# Autodesk Inventor assembly: BaseBotNoMod
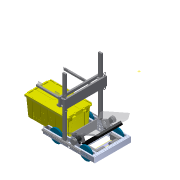
[picture p0: Inventor's stored thumbnail of the model, 180x180]
Saved by Autodesk Inventor 2015 (Build 190159000, 159)
## iProperties
Created: 2015-03-06
Part Number: BaseBotNoMod
Document SubType Name: Assembly
Designer: Kyle
Title: AM14U2 Long FIXED.STEP
Description: STEP AP214
Creation Date: 2015-01-13
Sending System: SolidWorks 2014
Preprocessor: SwSTEP 2.0
Author: Kyle
## Documents named in this file (23)
- E:\ReDesign\Project.iam
- E:\ReDesign\Imported Components\AM14U2+Long+FIXED\AM14U2 Half Long.iam
- E:\ReDesign\Wheel.ipt
- E:\ReDesign\Toughbox+Nano+All+Shafts+v2.iam
- E:\ReDesign\ControlBoard.ipt
- E:\ReDesign\LoadSlide.ipt
- E:\ReDesign\LoadSlideBracket.ipt
- E:\ReDesign\FrontSet.ipt
- E:\ReDesign\Imported Components\YELLOW_TOTEASM_ASM\YELLOW_TOTEASM_ASM.iam
- E:\ReDesign\ToteBasin.ipt
- E:\ReDesign\Lift Towers.ipt
- E:\ReDesign\PEG.iam
- E:\ReDesign\ArmAssembly.iam
- E:\ReDesign\RollerBearing.ipt
- E:\ReDesign\RollerBearingLong.ipt
- E:\ReDesign\ArmBacking.ipt
- E:\ReDesign\Imported Components\3014T974\3014T974.ipt
- E:\ReDesign\Imported Components\3112T330\3112T330.ipt
- E:\ReDesign\Imported Components\1x1tbar\1x1tbar.ipt
- E:\ReDesign\motorbracket.ipt
- E:\ReDesign\LongCap.iam
- E:\ReDesign\Imported Components\CIM Motor SW\CIM Motor SW.ipt
- E:\ReDesign\Spool.iam
## Components (43 placed, 23 different names)
1. AM14U2 Half Long_1 [sub-assembly] — Rotational:1, Mate:1, Mate:2, Mate:3, Rotational:3, Mate:6, Angle:2, Mate:9, Mate:10, Mate:18, Mate:19, Mate:23, Mate:30, Mate:31, Mate:32, Flush:2, Mate:78, Mate:79, Flush:7
2. AM14U2 Half Long_2 [sub-assembly] — Rotational:2, Mate:1, Mate:2, Mate:3, Rotational:4, Mate:4, Angle:1, Mate:8, Mate:20, Mate:21, Mate:26, Mate:27, Mate:28, Flush:1, Mate:76, Mate:77, Flush:6
3. Wheel:1 — Rotational:1, Mate:7
4. Wheel:2 — Rotational:2, Mate:5
5. Wheel:3 — Rotational:3
6. Wheel:4 — Rotational:4
7. Toughbox+Nano+All+Shafts+v2:1 [sub-assembly] — Mate:6, Mate:7, Angle:2
8. Toughbox+Nano+All+Shafts+v2:2 [sub-assembly] — Mate:4, Mate:5, Angle:1, Angle:3
9. ControlBoard:1 — Mate:8, Angle:3, Mate:9, Mate:10, Mate:11, Mate:12, Mate:13, Angle:4
10. LoadSlide:1 — Mate:11, Mate:12, Mate:13, Angle:4, Mate:14, Mate:22, Mate:24, Mate:85, Mate:86, Flush:12, Mate:89
11. LoadSlideBracket:1 — Mate:14, Mate:81, Mate:82, Mate:90
12. FrontSet:1 — Mate:18, Mate:19
13. FrontSet:2 — Mate:20, Mate:21
14. YELLOW_TOTEASM_ASM:1 [sub-assembly] — Mate:25
15. ToteBasin:1 — Mate:22, Mate:23, Mate:24, Mate:25
16. Lift Towers:1 — Mate:26, Mate:27, Mate:29, Tangent:2, Tangent:3, Tangent:5, Tangent:8, Mate:67, Angle:6
17. PEG:1 [sub-assembly] — Mate:28, Flush:1, Mate:29
18. Lift Towers:2 — Mate:30, Mate:31, Mate:33, Mate:57, Mate:58, Tangent:10, Tangent:11, Tangent:13, Tangent:16, Flush:3, Angle:5
19. PEG:2 [sub-assembly] — Mate:32, Flush:2, Mate:33
20. 3014T974:1 — Mate:70, Mate:71, Mate:72, Angle:5
21. 3014T974:2 — Mate:68, Mate:69, Mate:74, Angle:6
22. ArmAssembly:1 [sub-assembly] — Mate:57, Mate:58, Mate:59, Mate:60, Mate:61, Tangent:1, Tangent:4, Tangent:6, Mate:62, Tangent:7, Mate:63, Mate:64, Mate:65, Tangent:9, Tangent:12, Tangent:14, Mate:66, Tangent:15, Flush:4, Flush:5
23. RollerBearing:1 — Mate:59, Tangent:1, Tangent:2
24. RollerBearing:2 — Mate:60, Tangent:3, Tangent:4
25. RollerBearing:3 — Mate:61, Tangent:5, Tangent:6
26. RollerBearing:4 — Mate:64, Tangent:13, Tangent:14
27. RollerBearing:5 — Mate:65, Tangent:9, Tangent:10
28. RollerBearing:6 — Mate:63, Tangent:11, Tangent:12
29. RollerBearingLong:1 — Mate:62, Tangent:7, Tangent:8
30. RollerBearingLong:2 — Mate:66, Tangent:15, Tangent:16
31. ArmBacking:1 — Mate:67, Flush:3, Flush:4, Flush:5, Mate:68, Mate:69, Mate:70, Mate:71, Mate:73, Mate:75
32. 3112T330:2 — Mate:72, Mate:73
33. 3112T330:3 — Mate:74, Mate:75
34. 1x1tbar:1 — Mate:76, Mate:77, Flush:6
35. 1x1tbar:2 — Mate:78, Mate:79, Flush:7, Mate:80, Flush:8, Flush:9
36. LongCap:1 [sub-assembly] — Mate:80, Flush:8, Flush:9
37. motorbracket:2 — Mate:87, Mate:88, Mate:89, Flush:13, Mate:91
38. motorbracket:3 — Mate:81, Mate:82, Mate:83, Flush:10, Mate:90
39. CIM Motor SW:1 — Mate:83, Flush:10, Mate:84, Flush:11
40. Spool:1 [sub-assembly] — Mate:84, Flush:11
41. LoadSlideBracket:2 — Mate:85, Mate:86, Flush:12, Mate:87, Mate:88
42. CIM Motor SW:2 — Flush:13, Mate:91, Mate:92, Flush:14
43. Spool:2 [sub-assembly] — Mate:92, Flush:14
## Relationships (106: Mate 66, Tangent 16, Flush 14, Angle 6, RevoluteJoint 4)
- Rotational:1 [RevoluteJoint] (38.1 mm): AM14U2 Half Long_1 ↔ Wheel:1
- Rotational:2 [RevoluteJoint] (55.88 mm): AM14U2 Half Long_2 ↔ Wheel:2
- Mate:1: AM14U2 Half Long_1 ↔ AM14U2 Half Long_2
- Mate:2: AM14U2 Half Long_1 ↔ AM14U2 Half Long_2
- Mate:3: AM14U2 Half Long_1 ↔ AM14U2 Half Long_2
- Rotational:3 [RevoluteJoint] (57.15 mm): AM14U2 Half Long_1 ↔ Wheel:3
- Rotational:4 [RevoluteJoint] (55.88 mm): AM14U2 Half Long_2 ↔ Wheel:4
- Mate:4: AM14U2 Half Long_2 ↔ Toughbox+Nano+All+Shafts+v2:2
- Mate:5: Wheel:2 ↔ Toughbox+Nano+All+Shafts+v2:2
- Angle:1 (0 deg): AM14U2 Half Long_2 ↔ Toughbox+Nano+All+Shafts+v2:2
- Mate:6: AM14U2 Half Long_1 ↔ Toughbox+Nano+All+Shafts+v2:1
- Mate:7: Wheel:1 ↔ Toughbox+Nano+All+Shafts+v2:1
- Angle:2 (180 deg): AM14U2 Half Long_1 ↔ Toughbox+Nano+All+Shafts+v2:1
- Mate:8: AM14U2 Half Long_2 ↔ ControlBoard:1
- Angle:3 (134.9889 deg): Toughbox+Nano+All+Shafts+v2:2 ↔ ControlBoard:1
- Mate:9: AM14U2 Half Long_1 ↔ ControlBoard:1
- Mate:10: AM14U2 Half Long_1 ↔ ControlBoard:1
- Mate:11: ControlBoard:1 ↔ LoadSlide:1
- Mate:12 (44.45 mm): ControlBoard:1 ↔ LoadSlide:1
- Mate:13 (76.2 mm): ControlBoard:1 ↔ LoadSlide:1
- Angle:4 (68.7549 deg): ControlBoard:1 ↔ LoadSlide:1
- Mate:14: LoadSlide:1 ↔ LoadSlideBracket:1
- Mate:18: AM14U2 Half Long_1 ↔ FrontSet:1
- Mate:19: AM14U2 Half Long_1 ↔ FrontSet:1
- Mate:20: AM14U2 Half Long_2 ↔ FrontSet:2
- Mate:21: AM14U2 Half Long_2 ↔ FrontSet:2
- Mate:22: LoadSlide:1 ↔ ToteBasin:1
- Mate:23: AM14U2 Half Long_1 ↔ ToteBasin:1
- Mate:24: LoadSlide:1 ↔ ToteBasin:1
- Mate:25: YELLOW_TOTEASM_ASM:1 ↔ ToteBasin:1
- Mate:26: AM14U2 Half Long_2 ↔ Lift Towers:1
- Mate:27: AM14U2 Half Long_2 ↔ Lift Towers:1
- Mate:28: AM14U2 Half Long_2 ↔ PEG:1
- Flush:1 (-12.7 mm): AM14U2 Half Long_2 ↔ PEG:1
- Mate:29 (31.75 mm): Lift Towers:1 ↔ PEG:1
- Mate:30: AM14U2 Half Long_1 ↔ Lift Towers:2
- Mate:31: AM14U2 Half Long_1 ↔ Lift Towers:2
- Mate:32: AM14U2 Half Long_1 ↔ PEG:2
- Flush:2 (-12.7 mm): AM14U2 Half Long_1 ↔ PEG:2
- Mate:33 (31.75 mm): Lift Towers:2 ↔ PEG:2
- Mate:57: Lift Towers:2 ↔ ArmAssembly:1
- Mate:58 (38.1 mm): Lift Towers:2 ↔ ArmAssembly:1
- Mate:59: ArmAssembly:1 ↔ RollerBearing:1
- Mate:60: ArmAssembly:1 ↔ RollerBearing:2
- Mate:61: ArmAssembly:1 ↔ RollerBearing:3
- Tangent:1 (12.7 mm): ArmAssembly:1 ↔ RollerBearing:1
- Tangent:2: Lift Towers:1 ↔ RollerBearing:1
- Tangent:3: Lift Towers:1 ↔ RollerBearing:2
- Tangent:4 (12.7 mm): ArmAssembly:1 ↔ RollerBearing:2
- Tangent:5: Lift Towers:1 ↔ RollerBearing:3
- Tangent:6: ArmAssembly:1 ↔ RollerBearing:3
- Mate:62: ArmAssembly:1 ↔ RollerBearingLong:1
- Tangent:7: ArmAssembly:1 ↔ RollerBearingLong:1
- Tangent:8: Lift Towers:1 ↔ RollerBearingLong:1
- Mate:63: ArmAssembly:1 ↔ RollerBearing:6
- Mate:64: ArmAssembly:1 ↔ RollerBearing:4
- Mate:65: ArmAssembly:1 ↔ RollerBearing:5
- Tangent:9: ArmAssembly:1 ↔ RollerBearing:5
- Tangent:10: Lift Towers:2 ↔ RollerBearing:5
- Tangent:11: Lift Towers:2 ↔ RollerBearing:6
- Tangent:12 (12.7 mm): ArmAssembly:1 ↔ RollerBearing:6
- Tangent:13: Lift Towers:2 ↔ RollerBearing:4
- Tangent:14 (12.7 mm): ArmAssembly:1 ↔ RollerBearing:4
- Mate:66: ArmAssembly:1 ↔ RollerBearingLong:2
- Tangent:15: ArmAssembly:1 ↔ RollerBearingLong:2
- Tangent:16: Lift Towers:2 ↔ RollerBearingLong:2
- Mate:67: Lift Towers:1 ↔ ArmBacking:1
- Flush:3 (-38.1 mm): Lift Towers:2 ↔ ArmBacking:1
- Flush:4: ArmAssembly:1 ↔ ArmBacking:1
- Flush:5: ArmAssembly:1 ↔ ArmBacking:1
- Mate:68: 3014T974:2 ↔ ArmBacking:1
- Mate:69: 3014T974:2 ↔ ArmBacking:1
- Mate:70: 3014T974:1 ↔ ArmBacking:1
- Mate:71: 3014T974:1 ↔ ArmBacking:1
- Mate:72: 3014T974:1 ↔ 3112T330:2
- Mate:73: ArmBacking:1 ↔ 3112T330:2
- Mate:74: 3014T974:2 ↔ 3112T330:3
- Mate:75: ArmBacking:1 ↔ 3112T330:3
- Angle:5 (0 deg): Lift Towers:2 ↔ 3014T974:1
- Angle:6 (0 deg): Lift Towers:1 ↔ 3014T974:2
- Mate:76: AM14U2 Half Long_2 ↔ 1x1tbar:1
- Mate:77: AM14U2 Half Long_2 ↔ 1x1tbar:1
- Flush:6 (50.8 mm): AM14U2 Half Long_2 ↔ 1x1tbar:1
- Mate:78: AM14U2 Half Long_1 ↔ 1x1tbar:2
- Mate:79: AM14U2 Half Long_1 ↔ 1x1tbar:2
- Flush:7 (50.8 mm): AM14U2 Half Long_1 ↔ 1x1tbar:2
- Mate:80: 1x1tbar:2 ↔ LongCap:1
- Flush:8: 1x1tbar:2 ↔ LongCap:1
- Flush:9 (127 mm): 1x1tbar:2 ↔ LongCap:1
- Mate:81: LoadSlideBracket:1 ↔ motorbracket:3
- Mate:82: LoadSlideBracket:1 ↔ motorbracket:3
- Mate:83: motorbracket:3 ↔ CIM Motor SW:1
- Flush:10 (-76.2 mm): motorbracket:3 ↔ CIM Motor SW:1
- Mate:84: CIM Motor SW:1 ↔ Spool:1
- Flush:11: CIM Motor SW:1 ↔ Spool:1
- Mate:85: LoadSlide:1 ↔ LoadSlideBracket:2
- Mate:86 (-22.225 mm): LoadSlide:1 ↔ LoadSlideBracket:2
- Flush:12 (63.5 mm): LoadSlide:1 ↔ LoadSlideBracket:2
- Mate:87: motorbracket:2 ↔ LoadSlideBracket:2
- Mate:88: motorbracket:2 ↔ LoadSlideBracket:2
- Mate:89: LoadSlide:1 ↔ motorbracket:2
- Mate:90: LoadSlideBracket:1 ↔ motorbracket:3
- Flush:13 (13.0048 mm): motorbracket:2 ↔ CIM Motor SW:2
- Mate:91: motorbracket:2 ↔ CIM Motor SW:2
- Mate:92: CIM Motor SW:2 ↔ Spool:2
- Flush:14: CIM Motor SW:2 ↔ Spool:2
